# Autodesk Inventor assembly: Test tube rack
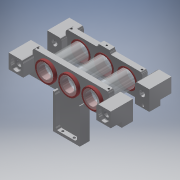
[picture p0: Inventor's stored thumbnail of the model, 180x180]
Saved by Autodesk Inventor 2017 (Build 210142000, 142)
## iProperties
Created: 2016-12-06
Part Number: Test tube rack
Document SubType Name: Assembly
Designer: qupec
Author: qupec
## Documents named in this file (9)
- C:\UMD\BPP\ROCKSAT X\star\CAD\Mechanical\Full payload assembly\Subsystems\Test Tube Rack\Test tube rack.iam
- C:\UMD\BPP\ROCKSAT X\star\CAD\Mechanical\Full payload assembly\Subsystems\Test Tube Rack\Test Tube.ipt
- C:\UMD\BPP\ROCKSAT X\star\CAD\Mechanical\Full payload assembly\Subsystems\Test Tube Rack\Test Tube Holder with Camera.ipt
- C:\UMD\BPP\ROCKSAT X\star\CAD\Mechanical\Full payload assembly\Subsystems\Test Tube Rack\Tube Rubber.ipt
- C:\UMD\BPP\ROCKSAT X\star\CAD\Mechanical\Full payload assembly\Subsystems\Test Tube Rack\Test Tube Holder.ipt
- C:\UMD\BPP\ROCKSAT X\star\CAD\Mechanical\Full payload assembly\Subsystems\Test Tube Rack\Bottom Test Tube Holder.ipt
- C:\UMD\BPP\ROCKSAT X\star\CAD\Mechanical\Full payload assembly\Subsystems\Test Tube Rack\Top Test Tube Holder.ipt
- C:\UMD\BPP\ROCKSAT X\star\CAD\Mechanical\Full payload assembly\Subsystems\Test Tube Rack\Linear Sleeve Bearing.ipt
- C:\UMD\BPP\ROCKSAT X\star\CAD\Mechanical\Spacer fot test tube rack.ipt
## Components (19 placed, 8 different names)
1. Test Tube Holder:1 — Mate:10, Mate:11, Mate:61, Mate:62, Mate:65, Mate:67, Mate:69, Mate:71, Mate:72, Mate:74, Mate:75
2. Bottom Test Tube Holder:1 — Mate:7, Mate:8, Mate:9, Mate:10, Mate:11, Mate:61
3. Tube Rubber:1 — Mate:3, Flush:6
4. Tube Rubber:2 — Mate:2, Flush:3
5. Tube Rubber:3 — Mate:4, Flush:5, Mate:8
6. Tube Rubber:4 — Mate:5, Flush:2, Mate:9
7. Tube Rubber:5 — Mate:1, Flush:4, Mate:7
8. Tube Rubber:6 — Mate:6, Flush:1
9. Test Tube:1 — Mate:5, Mate:6, Flush:1, Flush:2, Flush:13
10. Test Tube:2 — Mate:3, Mate:4, Flush:5, Flush:6, Flush:12
11. Test Tube:3 — Mate:1, Mate:2, Flush:3, Flush:4, Flush:11
12. Test Tube Holder with Camera:1 — Mate:26, Mate:27, Mate:60, Mate:63, Mate:64, Mate:66, Mate:68, Mate:70, Flush:14, Mate:73, Mate:76, Mate:77
13. Top Test Tube Holder:1 — Mate:26, Mate:27, Flush:11, Flush:12, Flush:13, Mate:60
14. Linear Sleeve Bearing:1 — Mate:63, Mate:68
15. Linear Sleeve Bearing:2 — Mate:62, Mate:69
16. Linear Sleeve Bearing:3 — Mate:65, Mate:67
17. Linear Sleeve Bearing:4 — Mate:64, Mate:66
18. Spacer fot test tube rack:1 — Mate:74, Mate:75, Mate:76
19. Spacer fot test tube rack:2 — Mate:71, Mate:72, Mate:73, Mate:77
## Relationships (41: Mate 31, Flush 10)
- Mate:1: Tube Rubber:5 ↔ Test Tube:3
- Mate:2: Tube Rubber:2 ↔ Test Tube:3
- Mate:3: Tube Rubber:1 ↔ Test Tube:2
- Mate:4: Tube Rubber:3 ↔ Test Tube:2
- Mate:5: Tube Rubber:4 ↔ Test Tube:1
- Mate:6: Tube Rubber:6 ↔ Test Tube:1
- Flush:1: Tube Rubber:6 ↔ Test Tube:1
- Flush:2: Tube Rubber:4 ↔ Test Tube:1
- Flush:3: Tube Rubber:2 ↔ Test Tube:3
- Flush:4: Tube Rubber:5 ↔ Test Tube:3
- Flush:5: Tube Rubber:3 ↔ Test Tube:2
- Flush:6: Tube Rubber:1 ↔ Test Tube:2
- Mate:7: Bottom Test Tube Holder:1 ↔ Tube Rubber:5
- Mate:8: Bottom Test Tube Holder:1 ↔ Tube Rubber:3
- Mate:9: Bottom Test Tube Holder:1 ↔ Tube Rubber:4
- Mate:10: Test Tube Holder:1 ↔ Bottom Test Tube Holder:1
- Mate:11: Test Tube Holder:1 ↔ Bottom Test Tube Holder:1
- Mate:26: Test Tube Holder with Camera:1 ↔ Top Test Tube Holder:1
- Mate:27: Test Tube Holder with Camera:1 ↔ Top Test Tube Holder:1
- Flush:11 (-3.175 mm): Test Tube:3 ↔ Top Test Tube Holder:1
- Flush:12 (-3.175 mm): Test Tube:2 ↔ Top Test Tube Holder:1
- Flush:13 (-3.175 mm): Test Tube:1 ↔ Top Test Tube Holder:1
- Mate:60: Test Tube Holder with Camera:1 ↔ Top Test Tube Holder:1
- Mate:61: Test Tube Holder:1 ↔ Bottom Test Tube Holder:1
- Mate:62: Test Tube Holder:1 ↔ Linear Sleeve Bearing:2
- Mate:63: Test Tube Holder with Camera:1 ↔ Linear Sleeve Bearing:1
- Mate:64: Test Tube Holder with Camera:1 ↔ Linear Sleeve Bearing:4
- Mate:65: Test Tube Holder:1 ↔ Linear Sleeve Bearing:3
- Mate:66: Test Tube Holder with Camera:1 ↔ Linear Sleeve Bearing:4
- Mate:67: Test Tube Holder:1 ↔ Linear Sleeve Bearing:3
- Mate:68: Test Tube Holder with Camera:1 ↔ Linear Sleeve Bearing:1
- Mate:69: Test Tube Holder:1 ↔ Linear Sleeve Bearing:2
- Mate:70: Test Tube Holder with Camera:1
- Flush:14: Test Tube Holder with Camera:1
- Mate:71: Test Tube Holder:1 ↔ Spacer fot test tube rack:2
- Mate:72: Test Tube Holder:1 ↔ Spacer fot test tube rack:2
- Mate:73: Test Tube Holder with Camera:1 ↔ Spacer fot test tube rack:2
- Mate:74: Test Tube Holder:1 ↔ Spacer fot test tube rack:1
- Mate:75: Test Tube Holder:1 ↔ Spacer fot test tube rack:1
- Mate:76: Test Tube Holder with Camera:1 ↔ Spacer fot test tube rack:1
- Mate:77: Test Tube Holder with Camera:1 ↔ Spacer fot test tube rack:2
